# Autodesk Inventor assembly: box
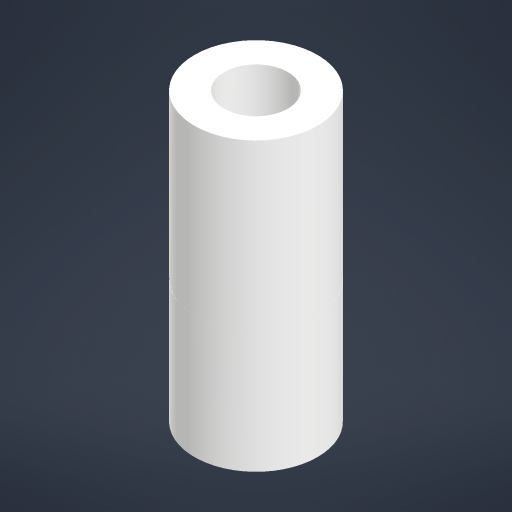
[picture p0: Inventor's stored thumbnail of the model, 512x512]
Saved by Autodesk Inventor 2024 (Build 280153000, 153)
## iProperties
Created: 2023-08-12
Part Number: box
Document SubType Name: Assembly
Designer: macbook
Author: macbook
## Documents named in this file (4)
- \\Mac\Home\Desktop\code\7899V-VRC-OVER-UNDER\Cad\VEX-CAD-Inventor-1.4.0\Motion\Spacers\box.iam
- \\Mac\Home\Desktop\code\7899V-VRC-OVER-UNDER\Cad\VEX-CAD-Inventor-1.4.0\Motion\Spacers\Spacer Nylon .313 OD\NSpacer .313 OD x .375.ipt
- \\Mac\Home\Desktop\code\7899V-VRC-OVER-UNDER\Cad\VEX-CAD-Inventor-1.4.0\Motion\Spacers\Spacer Nylon .313 OD.ipt
- \\Mac\Home\Desktop\code\7899V-VRC-OVER-UNDER\Cad\VEX-CAD-Inventor-1.4.0\Motion\Spacers\Spacer Nylon .313 OD\NSpacer .313 OD x .500.ipt
## Components (2 placed, 2 different names)
1. NSpacer .313 OD x .375:1 — Insert:1
2. NSpacer .313 OD x .500:2 — Insert:1
## Relationships (1: Insert 1)
- Insert:1: NSpacer .313 OD x .375:1 ↔ NSpacer .313 OD x .500:2
